# Autodesk Inventor assembly: assembly
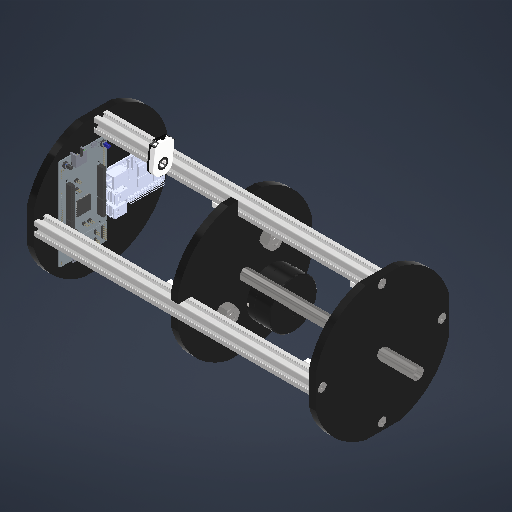
[picture p0: Inventor's stored thumbnail of the model, 512x512]
Saved by Autodesk Inventor 2027 (Build 310192000, 192)
## iProperties
Created: 2026-10-07
Part Number: assembly
Document SubType Name: Assembly
Designer: luca
Author: luca
## Documents named in this file (16)
- C:\Users\luca\Desktop\double_pendulum\RL-Rotary-Inverted-Double-Pendulum\CAD\assembly.iam
- C:\Users\luca\Desktop\double_pendulum\RL-Rotary-Inverted-Double-Pendulum\CAD\motor\L-7015-251029\2D3D\RMD-7015三维图\RMD-7015\RMD-7015.ipt
- C:\Users\luca\Desktop\double_pendulum\RL-Rotary-Inverted-Double-Pendulum\CAD\encoder\AMT102-D2048-I6350-S\3D\AMT102-D2048-I6350-S\AMT102-D2048-I6350-S.ipt
- C:\Users\luca\Desktop\double_pendulum\RL-Rotary-Inverted-Double-Pendulum\CAD\Electronics\RASPBERRY_PI_5\RASPBERRY_PI_5.ipt
- C:\Users\luca\Desktop\double_pendulum\RL-Rotary-Inverted-Double-Pendulum\CAD\Electronics\stm32\NUCLEO-F429ZI--3DModel-STEP-56544\NUCLEO-F429ZI--3DModel-STEP-56544.ipt
- C:\Users\luca\Desktop\double_pendulum\RL-Rotary-Inverted-Double-Pendulum\CAD\al-profil-20x20-drazka-6\al-profil-20x20-drazka-6.ipt
- C:\Users\luca\Desktop\double_pendulum\RL-Rotary-Inverted-Double-Pendulum\CAD\plate_lower.ipt
- C:\Users\luca\Desktop\double_pendulum\RL-Rotary-Inverted-Double-Pendulum\CAD\plate_middle.ipt
- C:\Users\luca\Desktop\double_pendulum\RL-Rotary-Inverted-Double-Pendulum\CAD\drive_shaft_center.ipt
- C:\Users\luca\Desktop\double_pendulum\RL-Rotary-Inverted-Double-Pendulum\CAD\plate_upper.ipt
- C:\Users\luca\Documents\Inventor\Content Center Files\R2027\de-DE\ASME ANSI B18.3.5M(2)\ASME_ANSI B18.3.5M - M6x40(2).ipt
- C:\Users\luca\Desktop\double_pendulum\RL-Rotary-Inverted-Double-Pendulum\CAD\motor_driveshaft.ipt
- C:\Users\luca\Desktop\double_pendulum\RL-Rotary-Inverted-Double-Pendulum\CAD\bearings\ucfl202.ipt
- C:\Users\luca\Desktop\double_pendulum\RL-Rotary-Inverted-Double-Pendulum\CAD\90_Deg_Profile\90_Deg_Profile.ipt
- C:\Users\luca\Documents\Inventor\Content Center Files\R2027\de-DE\AS 1420\AS 1420 - 1973 - M10 x 35.ipt
- C:\Users\luca\Documents\Inventor\Content Center Files\R2027\de-DE\AS 1252(3)\AS 1252 - M12.ipt
## Components (37 placed, 15 different names)
1. RMD-7015:1 — Passend:11, Passend:34, Passend:35
2. AMT102-D2048-I6350-S:1
3. RASPBERRY_PI_5:1 — Passend:7
4. NUCLEO-F429ZI--3DModel-STEP-56544:1 — Passend:6
5. plate_lower:1 — Passend:1, Passend:2, Passend:3, Passend:4, Passend:5, Winkel:1, Passend:6, Passend:7, Passend:17, Passend:19, Passend:26, Passend:27, Passend:28, Passend:29
6. plate_middle:1 — Passend:11, Passend:15, Passend:17, Passend:19, Winkel:2, Passend:40, Passend:42, Passend:46, Einfügen:5, Einfügen:6
7. drive_shaft_center:1 — Passend:15, Passend:39, Passend:41, Fluchtend:3
8. plate_upper:1 — Passend:18, Passend:20, Passend:21, Winkel:3, Passend:22, Passend:23, Passend:24, Passend:25, Passend:38, Passend:44
9. Senkkopfschraube mit gestanztem Innensechskant - Metrisch M6x40:1 — Passend:22
10. Senkkopfschraube mit gestanztem Innensechskant - Metrisch M6x40:2 — Passend:23
11. Senkkopfschraube mit gestanztem Innensechskant - Metrisch M6x40:3 — Passend:24
12. Senkkopfschraube mit gestanztem Innensechskant - Metrisch M6x40:4 — Passend:25
13. Senkkopfschraube mit gestanztem Innensechskant - Metrisch M6x40:5 — Passend:26
14. Senkkopfschraube mit gestanztem Innensechskant - Metrisch M6x40:6 — Passend:27
15. Senkkopfschraube mit gestanztem Innensechskant - Metrisch M6x40:7 — Passend:28
16. Senkkopfschraube mit gestanztem Innensechskant - Metrisch M6x40:8 — Passend:29
17. motor_driveshaft:1 — Passend:34, Passend:35
18. ucfl202:1 — Passend:40, Passend:41, Passend:46, Fluchtend:3, Einfügen:1, Einfügen:2, Einfügen:3, Einfügen:4
19. ucfl202:2 — Passend:38, Passend:39
20. AS 1420 - Metrisch M10 x 35:1 — Einfügen:1
21. AS 1420 - Metrisch M10 x 35:2 — Einfügen:2
22. AS 1420 - Metrisch M10 x 35:3 — Einfügen:3
23. AS 1420 - Metrisch M10 x 35:4 — Einfügen:4
24. AS 1252 - Metrisch M12:2 — Einfügen:5
25. AS 1252 - Metrisch M12:3 — Einfügen:6
26. al-profil-20x20-drazka-6:1 — Passend:4, Passend:5, Winkel:1, Passend:20, Passend:21
27. al-profil-20x20-drazka-6:2 — Passend:18, Winkel:2, Winkel:3, Passend:45, Fluchtend:2
28. al-profil-20x20-drazka-6:3
29. al-profil-20x20-drazka-6:4 — Fluchtend:1, Passend:43
30. 90_Deg_Profile:1 — Passend:42, Fluchtend:1, Passend:43
31. 90_Deg_Profile:2
32. 90_Deg_Profile:3
33. 90_Deg_Profile:4
34. 90_Deg_Profile:5 — Passend:44, Passend:45, Fluchtend:2
35. 90_Deg_Profile:6
36. 90_Deg_Profile:7
37. 90_Deg_Profile:8
## Component patterns: (4 elements, first: al-profil-20x20-drazka-6:1), (4 elements, first: 90_Deg_Profile:1), (4 elements, first: 90_Deg_Profile:5)
## Relationships (45: Mate 33, Insert 6, Angle 3, Flush 3)
- Passend:1 [Mate]: plate_lower:1
- Passend:2 [Mate]: plate_lower:1
- Passend:3 [Mate]: plate_lower:1
- Passend:4 [Mate]: plate_lower:1 ↔ al-profil-20x20-drazka-6:1
- Passend:5 [Mate]: plate_lower:1 ↔ al-profil-20x20-drazka-6:1
- Winkel:1 [Angle] (0 deg): plate_lower:1 ↔ al-profil-20x20-drazka-6:1
- Passend:6 [Mate]: NUCLEO-F429ZI--3DModel-STEP-56544:1 ↔ plate_lower:1
- Passend:7 [Mate]: RASPBERRY_PI_5:1 ↔ plate_lower:1
- Passend:11 [Mate]: RMD-7015:1 ↔ plate_middle:1
- Passend:15 [Mate]: plate_middle:1 ↔ drive_shaft_center:1
- Passend:17 [Mate] (200 mm): plate_lower:1 ↔ plate_middle:1
- Passend:18 [Mate]: plate_upper:1 ↔ al-profil-20x20-drazka-6:2
- Passend:19 [Mate]: plate_lower:1 ↔ plate_middle:1
- Winkel:2 [Angle] (0 deg): plate_middle:1 ↔ al-profil-20x20-drazka-6:2
- Passend:20 [Mate]: plate_upper:1 ↔ al-profil-20x20-drazka-6:1
- Passend:21 [Mate]: plate_upper:1 ↔ al-profil-20x20-drazka-6:1
- Winkel:3 [Angle] (0 deg): plate_upper:1 ↔ al-profil-20x20-drazka-6:2
- Passend:22 [Mate]: plate_upper:1 ↔ Senkkopfschraube mit gestanztem Innensechskant - Metrisch M6x40:1
- Passend:23 [Mate]: plate_upper:1 ↔ Senkkopfschraube mit gestanztem Innensechskant - Metrisch M6x40:2
- Passend:24 [Mate]: plate_upper:1 ↔ Senkkopfschraube mit gestanztem Innensechskant - Metrisch M6x40:3
- Passend:25 [Mate]: plate_upper:1 ↔ Senkkopfschraube mit gestanztem Innensechskant - Metrisch M6x40:4
- Passend:26 [Mate]: plate_lower:1 ↔ Senkkopfschraube mit gestanztem Innensechskant - Metrisch M6x40:5
- Passend:27 [Mate]: plate_lower:1 ↔ Senkkopfschraube mit gestanztem Innensechskant - Metrisch M6x40:6
- Passend:28 [Mate]: plate_lower:1 ↔ Senkkopfschraube mit gestanztem Innensechskant - Metrisch M6x40:7
- Passend:29 [Mate]: plate_lower:1 ↔ Senkkopfschraube mit gestanztem Innensechskant - Metrisch M6x40:8
- Passend:34 [Mate]: RMD-7015:1 ↔ motor_driveshaft:1
- Passend:35 [Mate]: RMD-7015:1 ↔ motor_driveshaft:1
- Passend:38 [Mate]: plate_upper:1 ↔ ucfl202:2
- Passend:39 [Mate]: drive_shaft_center:1 ↔ ucfl202:2
- Passend:40 [Mate]: plate_middle:1 ↔ ucfl202:1
- Passend:41 [Mate]: drive_shaft_center:1 ↔ ucfl202:1
- Passend:42 [Mate]: plate_middle:1 ↔ 90_Deg_Profile:1
- Fluchtend:1 [Flush]: al-profil-20x20-drazka-6:4 ↔ 90_Deg_Profile:1
- Passend:43 [Mate]: al-profil-20x20-drazka-6:4 ↔ 90_Deg_Profile:1
- Passend:44 [Mate]: plate_upper:1 ↔ 90_Deg_Profile:5
- Passend:45 [Mate]: al-profil-20x20-drazka-6:2 ↔ 90_Deg_Profile:5
- Fluchtend:2 [Flush]: al-profil-20x20-drazka-6:2 ↔ 90_Deg_Profile:5
- Passend:46 [Mate]: plate_middle:1 ↔ ucfl202:1
- Fluchtend:3 [Flush] (-5 mm): drive_shaft_center:1 ↔ ucfl202:1
- Einfügen:1 [Insert]: ucfl202:1 ↔ AS 1420 - Metrisch M10 x 35:1
- Einfügen:2 [Insert]: ucfl202:1 ↔ AS 1420 - Metrisch M10 x 35:2
- Einfügen:3 [Insert]: ucfl202:1 ↔ AS 1420 - Metrisch M10 x 35:3
- Einfügen:4 [Insert]: ucfl202:1 ↔ AS 1420 - Metrisch M10 x 35:4
- Einfügen:5 [Insert]: plate_middle:1 ↔ AS 1252 - Metrisch M12:2
- Einfügen:6 [Insert]: plate_middle:1 ↔ AS 1252 - Metrisch M12:3
